# Autodesk Inventor assembly: ForearmLeft
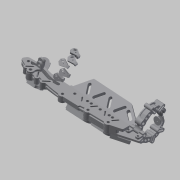
[picture p0: Inventor's stored thumbnail of the model, 180x180]
Saved by Autodesk Inventor 2015 SP1 (Build 190203100, 203)
## iProperties
Created: 2016-10-02
Part Number: ForearmLeft
Document SubType Name: Assembly
Designer: Val
Author: Val
## Documents named in this file (16)
- C:\Users\Val\Desktop\ExoGit\elysium-max-exoskeleton\src\Assemblies\ForearmLeft.iam
- C:\Users\Val\Desktop\ExoGit\elysium-max-exoskeleton\src\ForearmBase.ipt
- C:\Users\Val\Desktop\ExoGit\elysium-max-exoskeleton\src\ForearmInnerBase.ipt
- C:\Users\Val\Desktop\ExoGit\elysium-max-exoskeleton\src\ForearmLowerShockplateLeft.ipt
- C:\Users\Val\Desktop\ExoGit\elysium-max-exoskeleton\src\ForearmPistonConnector.ipt
- C:\Users\Val\Desktop\ExoGit\elysium-max-exoskeleton\src\ForearmUpperShockPlateLeft.ipt
- C:\Users\Val\Desktop\ExoGit\elysium-max-exoskeleton\src\LowerForearm.ipt
- C:\Users\Val\Desktop\ExoGit\elysium-max-exoskeleton\src\UpperForearmLeft.ipt
- C:\Users\Val\Desktop\ExoGit\elysium-max-exoskeleton\src\UpperForearmShockPlateConnectorLeft.ipt
- C:\Users\Val\Desktop\ExoGit\elysium-max-exoskeleton\src\ForearmClamp.ipt
- C:\Users\Val\Desktop\ExoGit\elysium-max-exoskeleton\src\ForearmClampHead.ipt
- C:\Users\Val\Desktop\ExoGit\elysium-max-exoskeleton\src\ForearmClampLink.ipt
- C:\Users\Val\Desktop\ExoGit\elysium-max-exoskeleton\src\ForearmCuffConnector.ipt
- C:\Users\Val\Desktop\ExoGit\elysium-max-exoskeleton\src\ElbowConnectorLeft.ipt
- C:\Users\Val\Desktop\ExoGit\elysium-max-exoskeleton\src\ElbowConnectorLinkLeft.ipt
- C:\Users\Val\Desktop\ExoGit\elysium-max-exoskeleton\src\ElbowConnectorUnderlinkLeft.ipt
## Components (22 placed, 15 different names)
1. ForearmBase:1 — Mate:2, Mate:3, Mate:4, Mate:5
2. ForearmInnerBase:1 — Mate:5, Mate:6, Mate:7, Mate:36, Mate:37
3. ForearmLowerShockplateLeft:1 — Mate:14, Mate:15, Mate:16
4. ForearmPistonConnector:1
5. ForearmUpperShockPlateLeft:1 — Mate:17, Mate:18, Mate:19
6. LowerForearm:1 — Mate:8, Mate:9, Mate:10, Mate:11, Mate:14, Mate:15, Mate:16, Mate:30, Mate:31, Mate:32, Mate:33, Mate:34
7. UpperForearmLeft:1 — Mate:2, Mate:3, Mate:4, Mate:6, Mate:7, Mate:8, Mate:9, Mate:10, Mate:12, Mate:13
8. UpperForearmShockPlateConnectorLeft:1 — Mate:11, Mate:12, Mate:13, Mate:17, Mate:18, Mate:19
9. ForearmClamp:1 — Flush:29, Mate:28, Rotational:2
10. ForearmClamp:2 — Mate:29, Flush:30, Rotational:1
11. ForearmClampHead:1 — Flush:29, Mate:28
12. ForearmClampHead:2 — Mate:29, Flush:30
13. ForearmClampLink:1 — Rotational:1, Rotational:2, Rotational:3, Mate:35
14. ForearmCuffConnector:1 — Rotational:3, Mate:30, Mate:31, Mate:32
15. ForearmCuffConnector:2 — Mate:33, Mate:34, Mate:35
16. ElbowConnectorLeft:1 — Mate:40, Mate:41
17. ElbowConnectorLinkLeft:1 — Mate:38, Mate:39, Angle:1, Mate:40, Mate:41
18. ElbowConnectorUnderlinkLeft:1 — Mate:36, Mate:37, Mate:38, Mate:39, Angle:1
19. ForearmPistonConnector:2
20. ForearmPistonConnector:3
21. ForearmPistonConnector:4
22. ForearmPistonConnector:5
## Relationships (38: Mate 32, RevoluteJoint 3, Flush 2, Angle 1)
- Mate:2: ForearmBase:1 ↔ UpperForearmLeft:1
- Mate:3: ForearmBase:1 ↔ UpperForearmLeft:1
- Mate:4: ForearmBase:1 ↔ UpperForearmLeft:1
- Mate:5: ForearmBase:1 ↔ ForearmInnerBase:1
- Mate:6: ForearmInnerBase:1 ↔ UpperForearmLeft:1
- Mate:7: ForearmInnerBase:1 ↔ UpperForearmLeft:1
- Mate:8: LowerForearm:1 ↔ UpperForearmLeft:1
- Mate:9: LowerForearm:1 ↔ UpperForearmLeft:1
- Mate:10: LowerForearm:1 ↔ UpperForearmLeft:1
- Mate:11: LowerForearm:1 ↔ UpperForearmShockPlateConnectorLeft:1
- Mate:12: UpperForearmLeft:1 ↔ UpperForearmShockPlateConnectorLeft:1
- Mate:13: UpperForearmLeft:1 ↔ UpperForearmShockPlateConnectorLeft:1
- Mate:14: ForearmLowerShockplateLeft:1 ↔ LowerForearm:1
- Mate:15: ForearmLowerShockplateLeft:1 ↔ LowerForearm:1
- Mate:16: ForearmLowerShockplateLeft:1 ↔ LowerForearm:1
- Mate:17: ForearmUpperShockPlateLeft:1 ↔ UpperForearmShockPlateConnectorLeft:1
- Mate:18: ForearmUpperShockPlateLeft:1 ↔ UpperForearmShockPlateConnectorLeft:1
- Mate:19: ForearmUpperShockPlateLeft:1 ↔ UpperForearmShockPlateConnectorLeft:1
- Flush:29 (3 mm): ForearmClamp:1 ↔ ForearmClampHead:1
- Mate:28: ForearmClamp:1 ↔ ForearmClampHead:1
- Mate:29: ForearmClamp:2 ↔ ForearmClampHead:2
- Flush:30 (3 mm): ForearmClamp:2 ↔ ForearmClampHead:2
- Rotational:1 [RevoluteJoint]: ForearmClamp:2 ↔ ForearmClampLink:1
- Rotational:2 [RevoluteJoint]: ForearmClamp:1 ↔ ForearmClampLink:1
- Rotational:3 [RevoluteJoint]: ForearmClampLink:1 ↔ ForearmCuffConnector:1
- Mate:30: LowerForearm:1 ↔ ForearmCuffConnector:1
- Mate:31: LowerForearm:1 ↔ ForearmCuffConnector:1
- Mate:32: LowerForearm:1 ↔ ForearmCuffConnector:1
- Mate:33: LowerForearm:1 ↔ ForearmCuffConnector:2
- Mate:34: LowerForearm:1 ↔ ForearmCuffConnector:2
- Mate:35: ForearmClampLink:1 ↔ ForearmCuffConnector:2
- Mate:36: ForearmInnerBase:1 ↔ ElbowConnectorUnderlinkLeft:1
- Mate:37: ForearmInnerBase:1 ↔ ElbowConnectorUnderlinkLeft:1
- Mate:38: ElbowConnectorLinkLeft:1 ↔ ElbowConnectorUnderlinkLeft:1
- Mate:39: ElbowConnectorLinkLeft:1 ↔ ElbowConnectorUnderlinkLeft:1
- Angle:1 (0 deg): ElbowConnectorLinkLeft:1 ↔ ElbowConnectorUnderlinkLeft:1
- Mate:40: ElbowConnectorLeft:1 ↔ ElbowConnectorLinkLeft:1
- Mate:41: ElbowConnectorLeft:1 ↔ ElbowConnectorLinkLeft:1
